# Autodesk Inventor assembly: Shooter Assembly
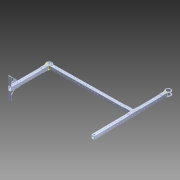
[picture p0: Inventor's stored thumbnail of the model, 180x180]
Saved by Autodesk Inventor 2014 (Build 180170000, 170)
## iProperties
Created: 2014-01-05
Part Number: Shooter Assembly
Document SubType Name: Assembly
Designer: Andrew Toennies
Mass: 581.2 g
Surface Area: 3707.46 cm^2
Volume: 214.465 cm^3
Density: 2.71 g/cm^3
Author: Andrew Toennies
## Documents named in this file (7)
- C:\Users\Andrew Toennies\Documents\GitHub\2014buildCAD\Shooter\Shooter Assembly.iam
- C:\Users\Andrew Toennies\Documents\GitHub\2014buildCAD\Shooter\Vex Pro 1x1 rectangular tubing 12 in length.ipt
- C:\Users\Andrew Toennies\Documents\GitHub\2014buildCAD\Shooter\Vex Pro End Bearing Mount.ipt
- C:\Users\Andrew Toennies\Documents\GitHub\2014buildCAD\Shooter\Vex Pro 1x1 rectangular tubing 27 in length.ipt
- C:\Users\Andrew Toennies\Documents\GitHub\2014buildCAD\Shooter\Vex Pro 1x1 rectangular tubing 24 in length.ipt
- C:\Users\Andrew Toennies\Documents\GitHub\2014buildCAD\Shooter\Vex Pro T gusset.ipt
- C:\Users\Andrew Toennies\Documents\GitHub\2014buildCAD\Shooter\Vex Pro Corner Gusset.ipt
## Components (11 placed, 6 different names)
1. Vex Pro 1x1 rectangular tubing 12 in length:1 — Insert:1, Insert:2, Insert:3, Insert:4, Flush:1, Insert:9, Insert:10, Insert:11, Insert:12
2. Vex Pro End Bearing Mount:1 — Insert:1, Insert:2, Mate:3
3. Vex Pro End Bearing Mount:2 — Insert:3, Insert:4
4. Vex Pro 1x1 rectangular tubing 27 in length:1 — Flush:1, Insert:5, Insert:6, Insert:7, Insert:8, Flush:2, Mate:2, Mate:3
5. Vex Pro 1x1 rectangular tubing 24 in length:1 — Flush:2, Mate:2, Insert:13, Insert:14, Insert:15, Insert:16
6. Vex Pro T gusset:1 — Insert:5, Insert:6
7. Vex Pro T gusset:2 — Insert:7, Insert:8
8. Vex Pro Corner Gusset:1 — Insert:9, Insert:10
9. Vex Pro Corner Gusset:2 — Insert:11, Insert:12
10. Vex Pro End Bearing Mount:3 — Insert:13, Insert:14
11. Vex Pro End Bearing Mount:4 — Insert:15, Insert:16
## Relationships (20: Insert 16, Flush 2, Mate 2)
- Insert:1: Vex Pro 1x1 rectangular tubing 12 in length:1 ↔ Vex Pro End Bearing Mount:1
- Insert:2: Vex Pro 1x1 rectangular tubing 12 in length:1 ↔ Vex Pro End Bearing Mount:1
- Insert:3: Vex Pro 1x1 rectangular tubing 12 in length:1 ↔ Vex Pro End Bearing Mount:2
- Insert:4: Vex Pro 1x1 rectangular tubing 12 in length:1 ↔ Vex Pro End Bearing Mount:2
- Flush:1: Vex Pro 1x1 rectangular tubing 12 in length:1 ↔ Vex Pro 1x1 rectangular tubing 27 in length:1
- Insert:5: Vex Pro 1x1 rectangular tubing 27 in length:1 ↔ Vex Pro T gusset:1
- Insert:6: Vex Pro 1x1 rectangular tubing 27 in length:1 ↔ Vex Pro T gusset:1
- Insert:7: Vex Pro 1x1 rectangular tubing 27 in length:1 ↔ Vex Pro T gusset:2
- Insert:8: Vex Pro 1x1 rectangular tubing 27 in length:1 ↔ Vex Pro T gusset:2
- Flush:2: Vex Pro 1x1 rectangular tubing 27 in length:1 ↔ Vex Pro 1x1 rectangular tubing 24 in length:1
- Mate:2: Vex Pro 1x1 rectangular tubing 27 in length:1 ↔ Vex Pro 1x1 rectangular tubing 24 in length:1
- Insert:9: Vex Pro 1x1 rectangular tubing 12 in length:1 ↔ Vex Pro Corner Gusset:1
- Insert:10: Vex Pro 1x1 rectangular tubing 12 in length:1 ↔ Vex Pro Corner Gusset:1
- Insert:11: Vex Pro 1x1 rectangular tubing 12 in length:1 ↔ Vex Pro Corner Gusset:2
- Insert:12: Vex Pro 1x1 rectangular tubing 12 in length:1 ↔ Vex Pro Corner Gusset:2
- Insert:13: Vex Pro 1x1 rectangular tubing 24 in length:1 ↔ Vex Pro End Bearing Mount:3
- Insert:14: Vex Pro 1x1 rectangular tubing 24 in length:1 ↔ Vex Pro End Bearing Mount:3
- Insert:15: Vex Pro 1x1 rectangular tubing 24 in length:1 ↔ Vex Pro End Bearing Mount:4
- Insert:16: Vex Pro 1x1 rectangular tubing 24 in length:1 ↔ Vex Pro End Bearing Mount:4
- Mate:3: Vex Pro End Bearing Mount:1 ↔ Vex Pro 1x1 rectangular tubing 27 in length:1
